# Autodesk Inventor assembly: dc Motor
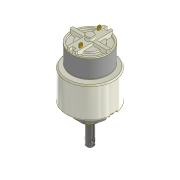
[picture p0: Inventor's stored thumbnail of the model, 180x180]
Saved by Autodesk Inventor 2020.3 (Build 243373000, 373)
## iProperties
Created: 2021-08-06
Part Number: dc Motor
Document SubType Name: Assembly
Designer: Suriyan.S
Author: Suriyan.S
## Documents named in this file (3)
- D:\MOP\Motor\Wheel_Motor\dc Motor.iam
- D:\MOP\Motor\Wheel_Motor\Nut.ipt
- D:\MOP\Motor\Wheel_Motor\Wheel Gear Motor.ipt
## Components (2 placed, 2 different names)
1. Nut:1 — Mate:1, Mate:2
2. Wheel Gear Motor:1 — Mate:1, Mate:2
## Relationships (2: Mate 2)
- Mate:1: Nut:1 ↔ Wheel Gear Motor:1
- Mate:2: Nut:1 ↔ Wheel Gear Motor:1
